# Autodesk Inventor assembly: Assembly
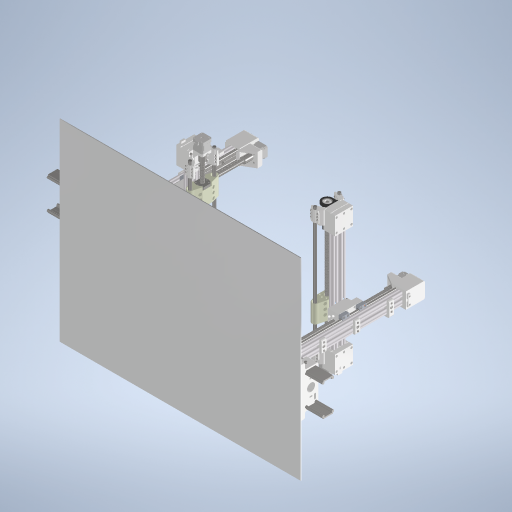
[picture p0: Inventor's stored thumbnail of the model, 512x512]
Saved by Autodesk Inventor 2024 (Build 280153000, 153)
## iProperties
Created: 2022-04-26
Part Number: Assembly
Document SubType Name: Assembly
Designer: mikoma
Author: mikoma
## Documents named in this file (6)
- D:\@home\mikoma\Dokumenty\DR\CartesianRobotsDigitalTwin\model\Workspaces\Obszar roboczy\assembly_v3\Assembly.iam
- D:\@home\mikoma\Dokumenty\DR\CartesianRobotsDigitalTwin\model\Workspaces\Obszar roboczy\assembly_v3\Y\Y.iam
- D:\@home\mikoma\Dokumenty\DR\CartesianRobotsDigitalTwin\model\Workspaces\Obszar roboczy\assembly_v3\Z\Z.iam
- D:\@home\mikoma\Dokumenty\DR\CartesianRobotsDigitalTwin\model\Workspaces\Obszar roboczy\assembly_v3\X\X.iam
- D:\@home\mikoma\Dokumenty\DR\CartesianRobotsDigitalTwin\model\Workspaces\Obszar roboczy\assembly_v3\C\Carriage.iam
- D:\@home\mikoma\Dokumenty\DR\CartesianRobotsDigitalTwin\model\Workspaces\Obszar roboczy\content\manipulatorSharedParts\aluminiumBase.ipt
## Components (9 placed, 5 different names)
1. aluminiumBase:1 — Zestawiające:11, Zestawiające:12, Równoległe:6, Równoległe:8, Równoległe:9
2. C [sub-assembly]
3. Z [sub-assembly] — Zestawiające:20, Zestawiające:21
4. X [sub-assembly] — Zestawiające:11, Równoległe:6, Zestawiające:19, Równoległe:7, Równoległe:8, Zestawiające:20, Zestawiające:21, Zestawiające:24
5. Y [sub-assembly]
6. Z:2 [sub-assembly] — Zestawiające:15, Zestawiające:16, Zestawiające:22, Zestawiające:23
7. Y:2 [sub-assembly] — Zestawiające:15, Zestawiające:16, Zestawiające:17, Zestawiające:18
8. C:2 [sub-assembly] — Zestawiające:17, Zestawiające:18
9. X:2 [sub-assembly] — Zestawiające:12, Równoległe:9, Zestawiające:22, Zestawiające:23, Zestawiające:24
## Relationships (21: Mate 15, Flush 5, Angle 1)
- [Flush]: X
- [Mate]: Z ↔ Y
- [Mate]: Z ↔ Y
- [Mate]: C ↔ Y
- [Angle] (0 deg): C ↔ Y
- Zestawiające:11 [Mate]: aluminiumBase:1 ↔ X
- Zestawiające:12 [Mate]: aluminiumBase:1 ↔ X:2
- Zestawiające:15 [Mate]: Z:2 ↔ Y:2
- Zestawiające:16 [Mate]: Z:2 ↔ Y:2
- Zestawiające:17 [Mate]: Y:2 ↔ C:2
- Zestawiające:18 [Mate]: Y:2 ↔ C:2
- Równoległe:6 [Flush]: aluminiumBase:1 ↔ X
- Zestawiające:19 [Mate]: X
- Równoległe:7 [Flush]: X
- Równoległe:8 [Flush] (215 mm): aluminiumBase:1 ↔ X
- Zestawiające:20 [Mate]: Z ↔ X
- Zestawiające:21 [Mate]: Z ↔ X
- Równoległe:9 [Flush]: aluminiumBase:1 ↔ X:2
- Zestawiające:22 [Mate]: Z:2 ↔ X:2
- Zestawiające:23 [Mate]: Z:2 ↔ X:2
- Zestawiające:24 [Mate] (-31 mm): X ↔ X:2
